# Autodesk Inventor assembly: Лестница вертикальная
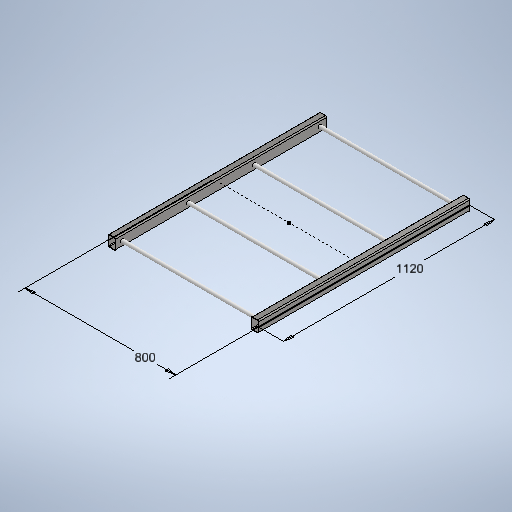
[picture p0: Inventor's stored thumbnail of the model, 512x512]
Saved by Autodesk Inventor 2025 (Build 290162010, 162A)
## iProperties
_SolveAssemblyDoc: Frame Generator Solve Assembly
_Version: 25.0.0
Created: 2024-09-17
Part Number: Лестница вертикальная
Document SubType Name: Assembly
Designer: pokla
Author: pokla
## Documents named in this file (4)
- C:\Users\pokla\Documents\Inventor\BSH_Beshkino_bio_tank\Лестница вертикальная.iam
- C:\Users\pokla\Documents\Inventor\BSH_Beshkino_bio_tank\Эскиз вертикальной лестницы.ipt
- C:\Users\pokla\Documents\Inventor\BSH_Beshkino_bio_tank\Лестница вертикальная\Frame\Frame 1726600970121.iam
- C:\Users\pokla\Documents\Inventor\BSH_Beshkino_bio_tank\пруток.ipt
## Components (6 placed, 3 different names)
1. Эскиз вертикальной лестницы:1
2. Frame 1726600970121:1 [sub-assembly] — Mate:1, Mate:2, Flush:1
3. пруток:1 — Mate:1, Mate:2, Flush:1
4. пруток:2
5. пруток:3
6. пруток:4
## Component patterns: (4 elements, first: пруток:1)
## Relationships (3: Mate 2, Flush 1)
- Mate:1: Frame 1726600970121:1 ↔ пруток:1
- Mate:2 (-35 mm): Frame 1726600970121:1 ↔ пруток:1
- Flush:1: Frame 1726600970121:1 ↔ пруток:1
